# Autodesk Inventor assembly: Assey_Course_C_v1
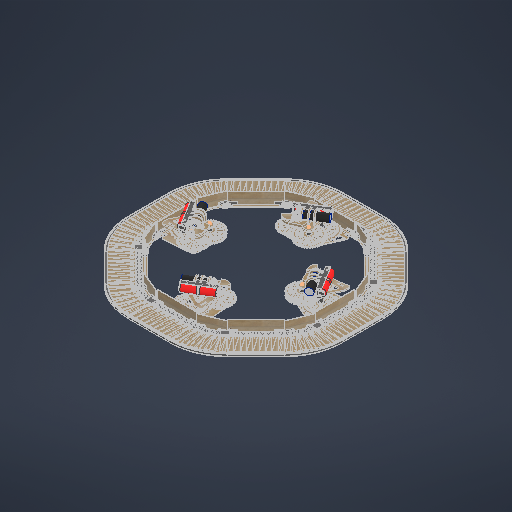
[picture p0: Inventor's stored thumbnail of the model, 512x512]
Saved by Autodesk Inventor 2026.3 (Build 303398000, 398)
## iProperties
Created: 2026-08-08
Part Number: Assey_Course_C_v1
Document SubType Name: Assembly
Designer: takuya
Author: takuya
## Documents named in this file (4)
- D:\model\D2_Conveyor_2026\2026\Assey_Course_C_v1.iam
- D:\model\D2_Conveyor_2026\power_module\Assy_power_module.iam
- D:\model\D2_Conveyor_2026\liniar_module\Assy_linear_module.iam
- D:\model\D2_Conveyor_2026\curve_module\Assy_curve_module.iam
## Components (20 placed, 3 different names)
1. Assy_linear_module:1 [sub-assembly] — メイト:1, メイト:2, メイト:3, メイト:4, フラッシュ:1, フラッシュ:2
2. Assy_curve_module:1 [sub-assembly] — メイト:2, メイト:4, フラッシュ:1, メイト:48, フラッシュ:28
3. Assy_curve_module:2 [sub-assembly] — メイト:1, メイト:3, フラッシュ:2, メイト:31, フラッシュ:18, メイト:47
4. Assy_linear_module:2 [sub-assembly]
5. Assy_curve_module:3 [sub-assembly] — メイト:50, メイト:52, フラッシュ:25
6. Assy_curve_module:4 [sub-assembly] — メイト:49, フラッシュ:27
7. Assy_linear_module:4 [sub-assembly]
8. Assy_curve_module:5 [sub-assembly] — メイト:43, メイト:45, フラッシュ:23
9. Assy_curve_module:6 [sub-assembly] — メイト:51, メイト:53, フラッシュ:26
10. Assy_linear_module:5 [sub-assembly]
11. Assy_curve_module:7 [sub-assembly] — メイト:30, フラッシュ:17, メイト:46
12. Assy_curve_module:8 [sub-assembly] — メイト:42, メイト:44, フラッシュ:24
13. Assy_linear_module:8 [sub-assembly] — メイト:30, メイト:31, 角度:1, フラッシュ:16, メイト:32, フラッシュ:17, フラッシュ:18, メイト:33, メイト:34, メイト:35, メイト:46, メイト:47
14. Assy_power_module:2 [sub-assembly] — 角度:1, フラッシュ:16, メイト:32, メイト:36, 角度:2
15. Assy_linear_module:10 [sub-assembly] — メイト:42, メイト:43, メイト:44, メイト:45, フラッシュ:23, フラッシュ:24, メイト:54, 角度:7
16. Assy_power_module:4 [sub-assembly] — メイト:61, 角度:11
17. Assy_linear_module:11 [sub-assembly] — メイト:50, メイト:51, メイト:52, メイト:53, フラッシュ:25, フラッシュ:26, メイト:55, 角度:8
18. Assy_power_module:5 [sub-assembly] — メイト:60, 角度:10
19. Assy_linear_module:12 [sub-assembly] — メイト:48, メイト:49, フラッシュ:27, フラッシュ:28, メイト:56, メイト:57, メイト:58
20. Assy_power_module:6 [sub-assembly] — メイト:59, 角度:9
## Relationships (80: Mate 50, Flush 20, Angle 10)
- メイト:1 [Mate]: Assy_linear_module:1 ↔ Assy_curve_module:2
- メイト:2 [Mate]: Assy_linear_module:1 ↔ Assy_curve_module:1
- メイト:3 [Mate]: Assy_linear_module:1 ↔ Assy_curve_module:2
- メイト:4 [Mate]: Assy_linear_module:1 ↔ Assy_curve_module:1
- フラッシュ:1 [Flush]: Assy_linear_module:1 ↔ Assy_curve_module:1
- フラッシュ:2 [Flush]: Assy_linear_module:1 ↔ Assy_curve_module:2
- [Mate]: Assy_linear_module:2 ↔ Assy_curve_module:4
- [Mate]: Assy_linear_module:2 ↔ Assy_curve_module:3
- [Mate]: Assy_linear_module:2 ↔ Assy_curve_module:4
- [Mate]: Assy_linear_module:2 ↔ Assy_curve_module:3
- [Flush]: Assy_linear_module:2 ↔ Assy_curve_module:3
- [Flush]: Assy_linear_module:2 ↔ Assy_curve_module:4
- [Mate]: Assy_linear_module:4 ↔ Assy_curve_module:6
- [Mate]: Assy_linear_module:4 ↔ Assy_curve_module:5
- [Mate]: Assy_linear_module:4 ↔ Assy_curve_module:6
- [Mate]: Assy_linear_module:4 ↔ Assy_curve_module:5
- [Flush]: Assy_linear_module:4 ↔ Assy_curve_module:5
- [Flush]: Assy_linear_module:4 ↔ Assy_curve_module:6
- [Mate]: Assy_linear_module:5 ↔ Assy_curve_module:8
- [Mate]: Assy_linear_module:5 ↔ Assy_curve_module:7
- [Mate]: Assy_linear_module:5 ↔ Assy_curve_module:8
- [Mate]: Assy_linear_module:5 ↔ Assy_curve_module:7
- [Flush]: Assy_linear_module:5 ↔ Assy_curve_module:7
- [Flush]: Assy_linear_module:5 ↔ Assy_curve_module:8
- メイト:30 [Mate]: Assy_curve_module:7 ↔ Assy_linear_module:8
- メイト:31 [Mate]: Assy_curve_module:2 ↔ Assy_linear_module:8
- 角度:1 [Angle] (0 deg): Assy_linear_module:8 ↔ Assy_power_module:2
- フラッシュ:16 [Flush]: Assy_linear_module:8 ↔ Assy_power_module:2
- メイト:32 [Mate]: Assy_linear_module:8 ↔ Assy_power_module:2
- フラッシュ:17 [Flush]: Assy_curve_module:7 ↔ Assy_linear_module:8
- フラッシュ:18 [Flush]: Assy_curve_module:2 ↔ Assy_linear_module:8
- メイト:33 [Mate]: Assy_linear_module:8
- メイト:34 [Mate]: Assy_linear_module:8
- メイト:35 [Mate]: Assy_linear_module:8
- メイト:36 [Mate]: Assy_power_module:2
- 角度:2 [Angle] (0 deg): Assy_power_module:2
- メイト:37 [Mate]
- [Angle] (0 deg): Assy_linear_module:10 ↔ Assy_power_module:4
- [Flush]: Assy_linear_module:10 ↔ Assy_power_module:4
- [Mate]: Assy_linear_module:10 ↔ Assy_power_module:4
- [Angle] (0 deg): Assy_linear_module:11 ↔ Assy_power_module:5
- [Flush]: Assy_linear_module:11 ↔ Assy_power_module:5
- [Mate]: Assy_linear_module:11 ↔ Assy_power_module:5
- [Angle] (0 deg): Assy_linear_module:12 ↔ Assy_power_module:6
- [Flush]: Assy_linear_module:12 ↔ Assy_power_module:6
- [Mate]: Assy_linear_module:12 ↔ Assy_power_module:6
- メイト:42 [Mate]: Assy_curve_module:8 ↔ Assy_linear_module:10
- メイト:43 [Mate]: Assy_curve_module:5 ↔ Assy_linear_module:10
- メイト:44 [Mate]: Assy_curve_module:8 ↔ Assy_linear_module:10
- メイト:45 [Mate]: Assy_curve_module:5 ↔ Assy_linear_module:10
- フラッシュ:23 [Flush]: Assy_curve_module:5 ↔ Assy_linear_module:10
- フラッシュ:24 [Flush]: Assy_curve_module:8 ↔ Assy_linear_module:10
- メイト:46 [Mate]: Assy_curve_module:7 ↔ Assy_linear_module:8
- メイト:47 [Mate]: Assy_curve_module:2 ↔ Assy_linear_module:8
- メイト:48 [Mate]: Assy_curve_module:1 ↔ Assy_linear_module:12
- メイト:49 [Mate]: Assy_curve_module:4 ↔ Assy_linear_module:12
- メイト:50 [Mate]: Assy_curve_module:3 ↔ Assy_linear_module:11
- メイト:51 [Mate]: Assy_curve_module:6 ↔ Assy_linear_module:11
- メイト:52 [Mate]: Assy_curve_module:3 ↔ Assy_linear_module:11
- メイト:53 [Mate]: Assy_curve_module:6 ↔ Assy_linear_module:11
- フラッシュ:25 [Flush]: Assy_curve_module:3 ↔ Assy_linear_module:11
- フラッシュ:26 [Flush]: Assy_curve_module:6 ↔ Assy_linear_module:11
- フラッシュ:27 [Flush]: Assy_curve_module:4 ↔ Assy_linear_module:12
- フラッシュ:28 [Flush]: Assy_curve_module:1 ↔ Assy_linear_module:12
- メイト:54 [Mate]: Assy_linear_module:10
- 角度:7 [Angle] (0 deg): Assy_linear_module:10
- メイト:55 [Mate]: Assy_linear_module:11
- 角度:8 [Angle] (0 deg): Assy_linear_module:11
- メイト:56 [Mate]: Assy_linear_module:12
- メイト:57 [Mate]: Assy_linear_module:12
- メイト:58 [Mate]: Assy_linear_module:12
- メイト:59 [Mate]: Assy_power_module:6
- 角度:9 [Angle] (0 deg): Assy_power_module:6
- メイト:60 [Mate]: Assy_power_module:5
- 角度:10 [Angle] (0 deg): Assy_power_module:5
- メイト:61 [Mate]: Assy_power_module:4
- 角度:11 [Angle] (0 deg): Assy_power_module:4
- メイト:62 [Mate]
- メイト:63 [Mate]
- メイト:64 [Mate]
## Named parameters: d6_d0 = 0 mm, d7_d1 = 0 mm, d8_d2 = 0 mm, d9_d3 = 0 mm, d10_d4 = 0 mm, d11_d5 = 0 mm, d12_d6_d0 = 0 mm, d13_d7_d1 = 0 mm, d14_d8_d2 = 0 mm, d15_d9_d3 = 0 mm, d16_d10_d4 = 0 mm, d17_d11_d5 = 0 mm, d18_d6_d0 = 0 mm, d19_d7_d1 = 0 mm, d20_d8_d2 = 0 mm, d21_d9_d3 = 0 mm, d22_d10_d4 = 0 mm, d23_d11_d5 = 0 mm, d62_d59_d48 = 0 deg, d63_d60_d49 = 0 mm, d64_d61_d50 = 0 mm, d65_d59_d48 = 0 deg, d66_d60_d49 = 0 mm, d67_d61_d50 = 0 mm, d68_d59_d48 = 0 deg, d69_d60_d49 = 0 mm, d70_d61_d50 = 0 mm
